# Autodesk Inventor assembly: XT-SM
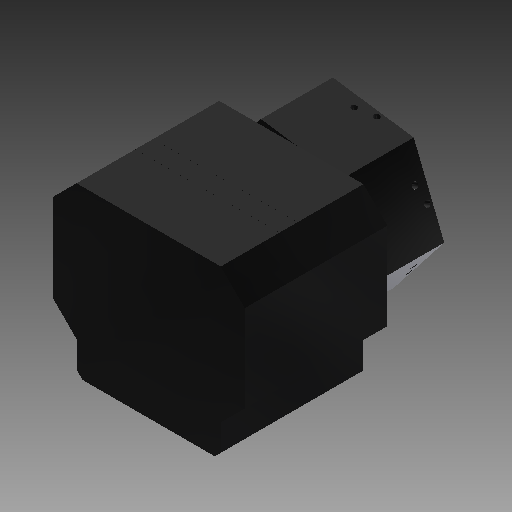
[picture p0: Inventor's stored thumbnail of the model, 512x512]
Saved by Autodesk Inventor 2017 SP1 (Build 210196100, 196)
## iProperties
Created: 2019-11-11
Part Number: XT-SM
Document SubType Name: Assembly
Designer: Dell
Author: Dell
## Documents named in this file (16)
- C:\Users\Zach\Documents\GitHub\tr2\Actuator 2.0\XT-SM.iam
- C:\Users\Zach\Documents\GitHub\tr2\Actuator 2.0\Custom Slewing.iam
- C:\Users\Zach\Documents\GitHub\tr2\Actuator 2.0\Series Elastic Gearbox 1.2\Series Elastic Gearbox 1.2.iam
- C:\Users\Zach\Documents\GitHub\tr2\Actuator 2.0\XT-SM-01.ipt
- C:\Users\Zach\Documents\GitHub\tr2\Actuator 2.0\XT-SM-02.ipt
- C:\Users\Zach\Documents\GitHub\tr2\Actuator 2.0\TS-40GZ495.ipt
- C:\Users\Zach\Documents\GitHub\tr2\Actuator 2.0\Actuator 2.0\Design Accelerator\Spur Gears3.iam
- C:\Users\Zach\Documents\GitHub\tr2\Actuator 2.0\Actuator 2.0\Design Accelerator\Spur Gears4.iam
- C:\Users\Zach\Documents\GitHub\tr2\Actuator 2.0\Actuator 2.0\Design Accelerator\Spur Gears5.iam
- C:\Users\Zach\Documents\GitHub\tr2\Actuator 2.0\XT-SM-03.ipt
- C:\Users\Zach\Documents\GitHub\tr2\Actuator 2.0\AEAT-6012.ipt
- C:\Users\Zach\Documents\GitHub\tr2\Actuator 2.0\AC09.ipt
- C:\Users\Zach\Documents\GitHub\tr2\Actuator 2.0\6201-2RS.ipt
- C:\Users\Zach\Documents\GitHub\tr2\Actuator 2.0\8mm Mounting Hub.ipt
- C:\Users\Zach\Documents\GitHub\tr2\Actuator 2.0\XT-SM-04.ipt
- C:\Users\Zach\Documents\GitHub\tr2\Actuator 2.0\XT-SM-05.ipt
## Components (17 placed, 13 different names)
1. Custom Slewing:1 [sub-assembly] — Mate:1, Mate:2, Mate:5, Mate:6, Mate:7, Mate:8, Mate:45, Mate:47
2. Series Elastic Gearbox 1.2:1 [sub-assembly] — Mate:5, Mate:9, Mate:10, Mate:14, Mate:15, Mate:16, Mate:18, Mate:19, Mate:20, Mate:21
3. XT-SM-01:1 — Mate:1, Mate:2, Mate:11, Mate:22, Mate:23, Mate:24, Mate:46, Angle:1, Mate:48
4. XT-SM-02:1 — Mate:6, Mate:7, Mate:8, Mate:9, Mate:10
5. TS-40GZ495:1 — Mate:11, Mate:17, Mate:40, Mate:41, Mate:42
6. Spur Gears:1 [sub-assembly] — Mate:14, Mate:15, Mate:16, Mate:17, Mate:18, Mate:43, Mate:44
7. Spur Gears:2 [sub-assembly] — Mate:19, Mate:20, Mate:21, Mate:22, Mate:25, Mate:33
8. Spur Gears:3 [sub-assembly] — Mate:23, Mate:26, Mate:34
9. XT-SM-03:1 — Mate:24, Mate:25, Mate:26, Mate:35, Mate:36, Mate:37, Mate:38, Mate:39, Mate:40, Mate:41, Mate:49, Flush:2, Flush:3
10. AEAT-6012:1
11. AEAT-6012:2
12. AC09:1 — Mate:37, Mate:38, Mate:39
13. 6201-2RS:1 — Mate:33, Mate:35
14. 6201-2RS:2 — Mate:34, Mate:36
15. 8mm Mounting Hub:1 — Mate:42, Mate:43, Mate:44
16. XT-SM-04:1 — Mate:47, Mate:48
17. XT-SM-05:1 — Mate:49, Flush:2, Flush:3
## Relationships (51: Mate 46, Flush 3, RelateRotation 1, Angle 1)
- Mate:1: Custom Slewing:1 ↔ XT-SM-01:1
- Mate:2: Custom Slewing:1 ↔ XT-SM-01:1
- Mate:5: Custom Slewing:1 ↔ Series Elastic Gearbox 1.2:1
- Mate:6: Custom Slewing:1 ↔ XT-SM-02:1
- Mate:7: Custom Slewing:1 ↔ XT-SM-02:1
- Mate:8: Custom Slewing:1 ↔ XT-SM-02:1
- Mate:9: Series Elastic Gearbox 1.2:1 ↔ XT-SM-02:1
- Mate:10: Series Elastic Gearbox 1.2:1 ↔ XT-SM-02:1
- Mate:11: XT-SM-01:1 ↔ TS-40GZ495:1
- [RelateRotation] (1.0714 ul): Spur Gears:1 ↔ Spur Gears:3
- [Mate] (1 mm): Spur Gears:1 ↔ Spur Gears:2
- [Flush]: Spur Gears:1 ↔ Spur Gears:3
- Mate:14: Series Elastic Gearbox 1.2:1 ↔ Spur Gears:1
- Mate:15: Series Elastic Gearbox 1.2:1 ↔ Spur Gears:1
- Mate:16: Series Elastic Gearbox 1.2:1 ↔ Spur Gears:1
- Mate:17: TS-40GZ495:1 ↔ Spur Gears:1
- Mate:18: Series Elastic Gearbox 1.2:1 ↔ Spur Gears:1
- Mate:19: Series Elastic Gearbox 1.2:1 ↔ Spur Gears:2
- Mate:20: Series Elastic Gearbox 1.2:1 ↔ Spur Gears:2
- Mate:21: Series Elastic Gearbox 1.2:1 ↔ Spur Gears:2
- Mate:22: XT-SM-01:1 ↔ Spur Gears:2
- Mate:23: XT-SM-01:1 ↔ Spur Gears:3
- Mate:24: XT-SM-01:1 ↔ XT-SM-03:1
- Mate:25: Spur Gears:2 ↔ XT-SM-03:1
- Mate:26: Spur Gears:3 ↔ XT-SM-03:1
- [Mate]: AEAT-6012:1 ↔ AC09:1
- [Mate]: AEAT-6012:1 ↔ AC09:1
- [Mate]: AEAT-6012:1 ↔ AC09:1
- [Mate]: AEAT-6012:2 ↔ AC09:1
- [Mate]: AEAT-6012:2 ↔ AC09:1
- [Mate]: AEAT-6012:2 ↔ AC09:1
- Mate:33: Spur Gears:2 ↔ 6201-2RS:1
- Mate:34: Spur Gears:3 ↔ 6201-2RS:2
- Mate:35: XT-SM-03:1 ↔ 6201-2RS:1
- Mate:36: XT-SM-03:1 ↔ 6201-2RS:2
- Mate:37: XT-SM-03:1 ↔ AC09:1
- Mate:38: XT-SM-03:1 ↔ AC09:1
- Mate:39: XT-SM-03:1 ↔ AC09:1
- Mate:40: TS-40GZ495:1 ↔ XT-SM-03:1
- Mate:41: TS-40GZ495:1 ↔ XT-SM-03:1
- Mate:42: TS-40GZ495:1 ↔ 8mm Mounting Hub:1
- Mate:43: Spur Gears:1 ↔ 8mm Mounting Hub:1
- Mate:44: Spur Gears:1 ↔ 8mm Mounting Hub:1
- Mate:45: Custom Slewing:1
- Mate:46: XT-SM-01:1
- Angle:1 (0 deg): XT-SM-01:1
- Mate:47: Custom Slewing:1 ↔ XT-SM-04:1
- Mate:48: XT-SM-01:1 ↔ XT-SM-04:1
- Mate:49: XT-SM-03:1 ↔ XT-SM-05:1
- Flush:2: XT-SM-03:1 ↔ XT-SM-05:1
- Flush:3: XT-SM-03:1 ↔ XT-SM-05:1
